# Autodesk Inventor assembly: E001-Chambre
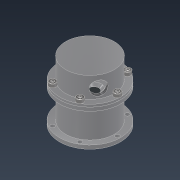
[picture p0: Inventor's stored thumbnail of the model, 180x180]
Saved by Autodesk Inventor 2021.3 (Build 253353000, 353)
## iProperties
Created: 2022-03-31
Part Number: E001-Chambre
Document SubType Name: Assembly
Designer: remi
Author: remi
## Documents named in this file (5)
- C:\Users\remi\OneDrive\Documents\Cours\05-HEVS\S2fb\mechanic\CCo\project\Compressor\E001-Chambre.iam
- C:\Users\remi\OneDrive\Documents\Cours\05-HEVS\S2fb\mechanic\CCo\project\Compressor\P002-Bati_chambre.ipt
- C:\Users\remi\OneDrive\Documents\Cours\05-HEVS\S2fb\mechanic\CCo\project\Compressor\P001-Couverture.ipt
- C:\Users\remi\OneDrive\Documents\Cours\05-HEVS\S2fb\mechanic\CCo\project\Compressor\P011-Chapeau_chambre.ipt
- C:\Users\remi\OneDrive\Documents\Inventor\Content Center Files\R2021\en-US\AS 1420\AS 1420 - 1973 - M3 x 6.ipt
## Components (9 placed, 4 different names)
1. P002-Bati_chambre:1 — Mate:1, Flush:1, Mate:2, Mate:3, Mate:4
2. P001-Couverture:1 — Mate:1, Flush:1
3. P011-Chapeau_chambre:1 — Mate:2, Mate:3, Mate:4, Insert:1, Insert:2, Insert:3, Insert:4, Insert:5, Insert:6
4. AS 1420 - Metric M3 x 6:1 — Insert:1
5. AS 1420 - Metric M3 x 6:2 — Insert:2
6. AS 1420 - Metric M3 x 6:3 — Insert:3
7. AS 1420 - Metric M3 x 6:4 — Insert:4
8. AS 1420 - Metric M3 x 6:5 — Insert:5
9. AS 1420 - Metric M3 x 6:6 — Insert:6
## Relationships (11: Insert 6, Mate 4, Flush 1)
- Mate:1: P002-Bati_chambre:1 ↔ P001-Couverture:1
- Flush:1: P002-Bati_chambre:1 ↔ P001-Couverture:1
- Mate:2: P002-Bati_chambre:1 ↔ P011-Chapeau_chambre:1
- Mate:3: P002-Bati_chambre:1 ↔ P011-Chapeau_chambre:1
- Mate:4: P002-Bati_chambre:1 ↔ P011-Chapeau_chambre:1
- Insert:1: P011-Chapeau_chambre:1 ↔ AS 1420 - Metric M3 x 6:1
- Insert:2: P011-Chapeau_chambre:1 ↔ AS 1420 - Metric M3 x 6:2
- Insert:3: P011-Chapeau_chambre:1 ↔ AS 1420 - Metric M3 x 6:3
- Insert:4: P011-Chapeau_chambre:1 ↔ AS 1420 - Metric M3 x 6:4
- Insert:5: P011-Chapeau_chambre:1 ↔ AS 1420 - Metric M3 x 6:5
- Insert:6: P011-Chapeau_chambre:1 ↔ AS 1420 - Metric M3 x 6:6
